# Autodesk Inventor assembly: Platform Assembly
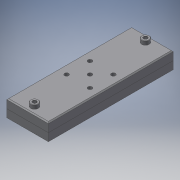
[picture p0: Inventor's stored thumbnail of the model, 180x180]
Saved by Autodesk Inventor 2019.4 (Build 234330000, 330)
## iProperties
Created: 2021-01-08
Part Number: Platform Assembly
Document SubType Name: Assembly
Designer: caleb
Author: caleb
## Documents named in this file (5)
- C:\Users\cfang\Desktop\nebraska-silicon-lab\CAD\ETL\Module Assembly\Picker Tool\Platform Assembly.iam
- C:\Users\cfang\Desktop\nebraska-silicon-lab\CAD\ETL\Module Assembly\Picker Tool\Platform A.ipt
- C:\Users\cfang\Desktop\nebraska-silicon-lab\CAD\ETL\Module Assembly\Picker Tool\Platform B.ipt
- C:\Users\cfang\Desktop\nebraska-silicon-lab\CAD\ETL\Module Assembly\Picker Tool\91292A113_TYPE 18-8 SS SOCKET HEAD CAP SCREW.ipt
- C:\Users\cfang\Desktop\nebraska-silicon-lab\CAD\ETL\Module Assembly\Picker Tool\1795N140_STATIC-DISSIPATIVE VACUUM CUP.ipt
## Components (6 placed, 4 different names)
1. Platform A:1 — Mate:1, Flush:1, Flush:2, Insert:1, Insert:2
2. Platform B:1 — Mate:1, Flush:1, Flush:2, Insert:3, Insert:4
3. 91292A113_TYPE 18-8 SS SOCKET HEAD CAP SCREW:1 — Insert:1
4. 91292A113_TYPE 18-8 SS SOCKET HEAD CAP SCREW:2 — Insert:2
5. 1795N140_STATIC-DISSIPATIVE VACUUM CUP:1 — Insert:3
6. 1795N140_STATIC-DISSIPATIVE VACUUM CUP:2 — Insert:4
## Relationships (7: Insert 4, Flush 2, Mate 1)
- Mate:1: Platform A:1 ↔ Platform B:1
- Flush:1: Platform A:1 ↔ Platform B:1
- Flush:2: Platform A:1 ↔ Platform B:1
- Insert:1: Platform A:1 ↔ 91292A113_TYPE 18-8 SS SOCKET HEAD CAP SCREW:1
- Insert:2: Platform A:1 ↔ 91292A113_TYPE 18-8 SS SOCKET HEAD CAP SCREW:2
- Insert:3: Platform B:1 ↔ 1795N140_STATIC-DISSIPATIVE VACUUM CUP:1
- Insert:4: Platform B:1 ↔ 1795N140_STATIC-DISSIPATIVE VACUUM CUP:2
